# Autodesk Inventor assembly: ChipMountAss
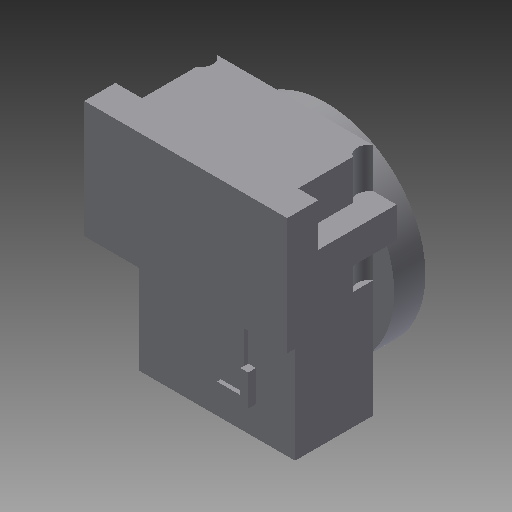
[picture p0: Inventor's stored thumbnail of the model, 512x512]
Saved by Autodesk Inventor 2019 (Build 230136000, 136)
## iProperties
Created: 2019-05-21
Part Number: ChipMountAss
Document SubType Name: Assembly
Designer: aorfi
Author: aorfi
## Documents named in this file (4)
- C:\Users\aorfi\OneDrive\Documents\IQC\ChipMountAssembly.iam
- C:\Users\aorfi\OneDrive\Documents\IQC\CustomParts\ChipMount.ipt
- C:\Users\aorfi\OneDrive\Documents\IQC\CustomParts\Chip.ipt
- C:\Users\aorfi\OneDrive\Documents\IQC\CustomParts\Cover.ipt
## Components (3 placed, 3 different names)
1. ChipMount:1 — Flush:1, Flush:2, Flush:3, Mate:1, Mate:2, Mate:3, Mate:6
2. Chip:1 — Mate:1, Mate:2, Mate:3
3. Cover:1 — Mate:5, Mate:6
## Relationships (8: Mate 5, Flush 3)
- Flush:1: ChipMount:1
- Flush:2: ChipMount:1
- Flush:3: ChipMount:1
- Mate:1: ChipMount:1 ↔ Chip:1
- Mate:2: ChipMount:1 ↔ Chip:1
- Mate:3: ChipMount:1 ↔ Chip:1
- Mate:5: Cover:1
- Mate:6: ChipMount:1 ↔ Cover:1
